# Autodesk Inventor assembly: assembly
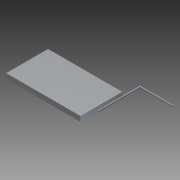
[picture p0: Inventor's stored thumbnail of the model, 180x180]
Saved by Autodesk Inventor 2014 (Build 180170000, 170)
## iProperties
Created: 2014-03-21
Part Number: assembly
Document SubType Name: Assembly
Designer: joe_000
Author: joe_000
## Documents named in this file (4)
- C:\dev\camera-multitouch\mounting-bracket\assembly.iam
- C:\dev\camera-multitouch\mounting-bracket\tv.ipt
- C:\dev\camera-multitouch\mounting-bracket\arm-vertical.ipt
- C:\dev\camera-multitouch\mounting-bracket\arm-horizontal.ipt
## Components (3 placed, 3 different names)
1. tv:1 — Insert:1, Insert:2
2. arm-vertical:1 — Insert:1, Insert:2, Flush:1, Flush:2, Mate:1
3. arm-horizontal:1 — Flush:1, Flush:2, Mate:1
## Relationships (5: Insert 2, Flush 2, Mate 1)
- Insert:1: tv:1 ↔ arm-vertical:1
- Insert:2: tv:1 ↔ arm-vertical:1
- Flush:1: arm-vertical:1 ↔ arm-horizontal:1
- Flush:2: arm-vertical:1 ↔ arm-horizontal:1
- Mate:1: arm-vertical:1 ↔ arm-horizontal:1
